# Autodesk Inventor assembly: Mold Design1
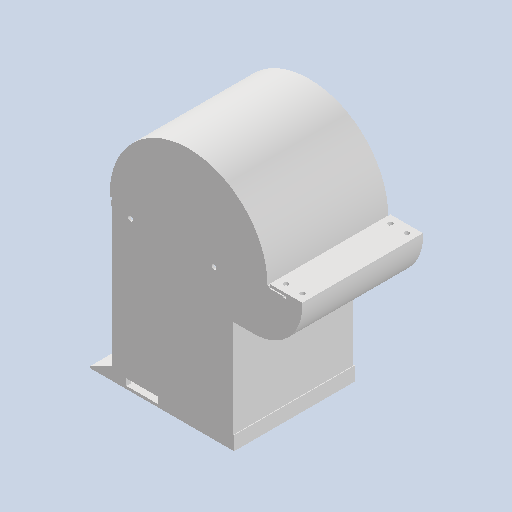
[picture p0: Inventor's stored thumbnail of the model, 512x512]
Saved by Autodesk Inventor 2025 (Build 290162000, 162)
## iProperties
Created: 2025-08-28
Part Number: Mold Design1
Document SubType Name: Assembly
Designer: Pravoslav
Author: Pravoslav
## Documents named in this file (6)
- D:\Škola\VUT\Igem\šachta\taker\dávkovanie\konnst\Mold Design1.iam
- D:\Škola\VUT\Igem\šachta\taker\dávkovanie\konnst\bottom.ipt
- D:\Škola\VUT\Igem\šachta\taker\dávkovanie\konnst\Low.ipt
- D:\Škola\VUT\Igem\šachta\taker\dávkovanie\konnst\Holder.ipt
- D:\Škola\VUT\Igem\šachta\taker\dávkovanie\konnst\coupol.ipt
- D:\Škola\VUT\Igem\šachta\taker\dávkovanie\konnst\cap.ipt
## Components (5 placed, 5 different names)
1. bottom:1 — Mate:1
2. Low:1 — Mate:1, Mate:2
3. Holder:1 — Mate:2, Mate:3, Mate:4
4. coupol:1 — Mate:3
5. cap:1 — Mate:4
## Relationships (4: Mate 4)
- Mate:1: bottom:1 ↔ Low:1
- Mate:2: Low:1 ↔ Holder:1
- Mate:3: Holder:1 ↔ coupol:1
- Mate:4: Holder:1 ↔ cap:1
